# Autodesk Inventor assembly: OCEAN-Pocitadlo
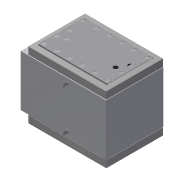
[picture p0: Inventor's stored thumbnail of the model, 180x180]
Saved by Autodesk Inventor 2017 (Build 210142000, 142)
## iProperties
Created: 2014-02-17
Part Number: OCEAN-Pocitadlo
Document SubType Name: Assembly
Designer: Евтушенко
Author: Евтушенко
## Documents named in this file (8)
- D:\ИНИТ\STEP файлы\Колонки\OCEAN-36-WAVE\OCEAN-Pocitadlo.iam
- D:\ИНИТ\STEP файлы\Колонки\OCEAN-36-WAVE\1556-211b.iam
- D:\ИНИТ\STEP файлы\Колонки\OCEAN-36-WAVE\M003372.ipt
- D:\ИНИТ\STEP файлы\Колонки\OCEAN-36-WAVE\M003373.ipt
- D:\ИНИТ\STEP файлы\Колонки\OCEAN-36-WAVE\2684-411.ipt
- D:\ИНИТ\STEP файлы\Колонки\OCEAN-36-WAVE\Sroub_DIN_923_M4x6.ipt
- D:\ИНИТ\STEP файлы\Колонки\OCEAN-36-WAVE\2795-411.ipt
- D:\ИНИТ\Разработка\Терминалы\Info Media Ocean - IO\02 - Конструктив\IO.02.00.00-07.iam
## Components (15 placed, 7 different names)
1. 1556-211b:1 [sub-assembly] — Совмещение:1, Заподлицо:1, Угол:1, Совмещение:2, Угол:2, Заподлицо:2
2. M003372:1
3. M003373:1
4. M003372:2
5. M003373:2
6. 2684-411:1
7. 2684-411:2
8. Sroub_DIN_923_M4x6:1
9. 2795-411:1
10. 2795-411:2
11. Sroub_DIN_923_M4x6:2
12. Sroub_DIN_923_M4x6:3
13. Sroub_DIN_923_M4x6:4
14. IO.02.00.00-07:1 [sub-assembly] — Совмещение:1, Заподлицо:1, Угол:1
15. IO.02.00.00-07:2 [sub-assembly] — Совмещение:2, Угол:2, Заподлицо:2
## Relationships (6: Mate 2, Flush 2, Angle 2)
- Совмещение:1 [Mate]: 1556-211b:1 ↔ IO.02.00.00-07:1
- Заподлицо:1 [Flush]: 1556-211b:1 ↔ IO.02.00.00-07:1
- Угол:1 [Angle] (0 deg): 1556-211b:1 ↔ IO.02.00.00-07:1
- Совмещение:2 [Mate]: 1556-211b:1 ↔ IO.02.00.00-07:2
- Угол:2 [Angle] (0 deg): 1556-211b:1 ↔ IO.02.00.00-07:2
- Заподлицо:2 [Flush]: 1556-211b:1 ↔ IO.02.00.00-07:2
